# Autodesk Inventor assembly: power_supply
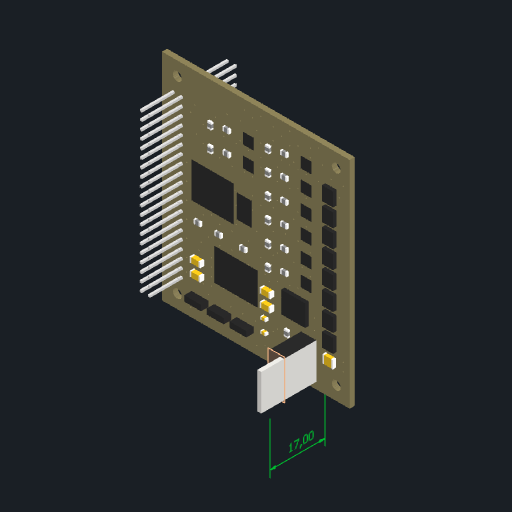
[picture p0: Inventor's stored thumbnail of the model, 512x512]
Saved by Autodesk Inventor 2023 (Build 270158030, 158C)
## iProperties
Created: 2022-07-11
Part Number: power_supply
Document SubType Name: Assembly
Designer: Administrator
Title: power_supply v2
Author: Administrator
## Documents named in this file (4)
- C:\Users\norbe\Repozytoria\NormalMapScanner\3D_modeling\power_supply_pcb\power_supply.iam
- C:\Users\norbe\Repozytoria\NormalMapScanner\3D_modeling\power_supply_pcb\Board.ipt
- C:\Users\norbe\Repozytoria\NormalMapScanner\3D_modeling\power_supply_pcb\Packages.iam
- C:\Users\norbe\Repozytoria\NormalMapScanner\3D_modeling\power_supply_pcb\raspberry_goldpins_2x40\Pin Header 20x2 TH Pitch 2.54mm v1.iam
## Components (3 placed, 3 different names)
1. Board:1 — Mate:1, Tangent:1, Tangent:2
2. Packages:1 [sub-assembly]
3. Pin Header 20x2 TH Pitch 2.54mm v1:1 [sub-assembly] — Mate:1, Tangent:1, Tangent:2
## Relationships (3: Tangent 2, Mate 1)
- Mate:1: Board:1 ↔ Pin Header 20x2 TH Pitch 2.54mm v1:1
- Tangent:1: Board:1 ↔ Pin Header 20x2 TH Pitch 2.54mm v1:1
- Tangent:2: Board:1 ↔ Pin Header 20x2 TH Pitch 2.54mm v1:1
